# Autodesk Inventor assembly: Default Motor Testbench Mk4
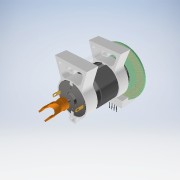
[picture p0: Inventor's stored thumbnail of the model, 180x180]
Saved by Autodesk Inventor 2018 (Build 220112000, 112)
## iProperties
Created: 2018-01-25
Part Number: Default Motor Testbench Mk4
Document SubType Name: Assembly
Designer: Moochster
Author: Moochster
## Documents named in this file (9)
- C:\Users\Moochster\OneDrive\Documents\2018 UBC\ELEC 391\Controller\CAD\Default Motor Testbench Mk4.iam
- C:\Users\Moochster\OneDrive\Documents\2018 UBC\ELEC 391\Controller\CAD\JD5B-2655W-R.ipt
- C:\Users\Moochster\OneDrive\Documents\2018 UBC\ELEC 391\Controller\CAD\Encoder Wheel (G16).ipt
- C:\Users\Moochster\OneDrive\Documents\2018 UBC\ELEC 391\Controller\CAD\Laser Mount.ipt
- C:\Users\Moochster\OneDrive\Documents\2018 UBC\ELEC 391\Controller\CAD\Motor Reversed Mount.ipt
- C:\Users\Moochster\OneDrive\Documents\2018 UBC\ELEC 391\Controller\CAD\Motor Reversed Mount Midsection.ipt
- C:\Users\Moochster\OneDrive\Documents\2018 UBC\ELEC 391\Controller\CAD\Motor Mount Slot Lock.ipt
- C:\Users\Moochster\OneDrive\Documents\2018 UBC\ELEC 391\Controller\CAD\GP1A52HRJ00F (Large slot detector).ipt
- C:\Users\Moochster\OneDrive\Documents\2018 UBC\ELEC 391\Controller\CAD\Slot Detector Holder.ipt
## Components (10 placed, 8 different names)
1. JD5B-2655W-R:1 — Mate:1, Mate:2, Mate:3, Mate:4, Mate:5, Flush:2, Mate:6, Mate:13
2. Encoder Wheel (G16):1 — Mate:1, Mate:12, Mate:13, Angle:3
3. Laser Mount:1 — Mate:2, Mate:4, Angle:3
4. Motor Reversed Mount:1 — Mate:5, Angle:1, Flush:2, Flush:3, Mate:7, Mate:8, Mate:9, Mate:10
5. Motor Reversed Mount Midsection:1 — Mate:6, Flush:3
6. Motor Mount Slot Lock:1 — Mate:7, Mate:8
7. Motor Mount Slot Lock:2 — Mate:9, Mate:10
8. GP1A52HRJ00F (Large slot detector):1 — Mate:11, Flush:4, Flush:5, Angle:2, Mate:14, Mate:15
9. GP1A52HRJ00F (Large slot detector):2 — Mate:11, Flush:4, Flush:5, Mate:12
10. Slot Detector Holder:1 — Mate:14, Mate:15
## Relationships (22: Mate 15, Flush 4, Angle 3)
- Mate:1: JD5B-2655W-R:1 ↔ Encoder Wheel (G16):1
- Mate:2: JD5B-2655W-R:1 ↔ Laser Mount:1
- Mate:3: JD5B-2655W-R:1
- Mate:4 (4 mm): JD5B-2655W-R:1 ↔ Laser Mount:1
- Mate:5: JD5B-2655W-R:1 ↔ Motor Reversed Mount:1
- Angle:1 (0 deg): Motor Reversed Mount:1
- Flush:2: JD5B-2655W-R:1 ↔ Motor Reversed Mount:1
- Mate:6: JD5B-2655W-R:1 ↔ Motor Reversed Mount Midsection:1
- Flush:3: Motor Reversed Mount:1 ↔ Motor Reversed Mount Midsection:1
- Mate:7 (0.15 mm): Motor Reversed Mount:1 ↔ Motor Mount Slot Lock:1
- Mate:8 (0.15 mm): Motor Reversed Mount:1 ↔ Motor Mount Slot Lock:1
- Mate:9 (0.15 mm): Motor Reversed Mount:1 ↔ Motor Mount Slot Lock:2
- Mate:10 (0.15 mm): Motor Reversed Mount:1 ↔ Motor Mount Slot Lock:2
- Mate:11 (0.1 mm): GP1A52HRJ00F (Large slot detector):1 ↔ GP1A52HRJ00F (Large slot detector):2
- Flush:4: GP1A52HRJ00F (Large slot detector):1 ↔ GP1A52HRJ00F (Large slot detector):2
- Flush:5: GP1A52HRJ00F (Large slot detector):1 ↔ GP1A52HRJ00F (Large slot detector):2
- Mate:12 (0.75 mm): Encoder Wheel (G16):1 ↔ GP1A52HRJ00F (Large slot detector):2
- Angle:2 (0 deg): GP1A52HRJ00F (Large slot detector):1
- Mate:13 (1 mm): JD5B-2655W-R:1 ↔ Encoder Wheel (G16):1
- Angle:3 (0 deg): Encoder Wheel (G16):1 ↔ Laser Mount:1
- Mate:14 (0.075 mm): GP1A52HRJ00F (Large slot detector):1 ↔ Slot Detector Holder:1
- Mate:15 (0.075 mm): GP1A52HRJ00F (Large slot detector):1 ↔ Slot Detector Holder:1
